# Autodesk Inventor assembly: CubeLift
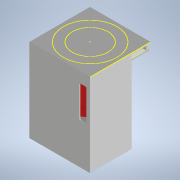
[picture p0: Inventor's stored thumbnail of the model, 180x180]
Saved by Autodesk Inventor 2020 (Build 240168000, 168)
## iProperties
Created: 2020-05-15
Part Number: CubeLift
Document SubType Name: Assembly
Designer: jurre
Author: jurre
## Documents named in this file (5)
- C:\Users\jurre\Documents\CubeLift\CubeLift.iam
- C:\Users\jurre\Documents\CubeLift\Stepper.ipt
- C:\Users\jurre\Documents\CubeLift\Drum.ipt
- C:\Users\jurre\Downloads\bearings-608zz-80018-1.snapshot.1\608zz (80018).ipt
- C:\Users\jurre\Documents\CubeLift\Mount.ipt
## Components (4 placed, 4 different names)
1. Stepper:1 — Flush:1, Rotational:2
2. Drum:1 — Flush:1, Rotational:1, Rotational:2, Flush:2, Flush:3
3. 608zz (80018):1 — Rotational:1
4. Mount:1 — Flush:2, Flush:3
## Relationships (5: Flush 3, RevoluteJoint 2)
- Flush:1: Stepper:1 ↔ Drum:1
- Rotational:1 [RevoluteJoint]: Drum:1 ↔ 608zz (80018):1
- Rotational:2 [RevoluteJoint]: Stepper:1 ↔ Drum:1
- Flush:2: Drum:1 ↔ Mount:1
- Flush:3: Drum:1 ↔ Mount:1
